# Autodesk Inventor assembly: EngranajesPegados
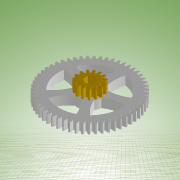
[picture p0: Inventor's stored thumbnail of the model, 180x180]
Saved by Autodesk Inventor 2022 (Build 260153000, 153)
## iProperties
Created: 2022-03-08
Part Number: EngranajesPegados
Document SubType Name: Assembly
Designer: Marco
Author: Marco
## Documents named in this file (3)
- C:\Users\steff\Desktop\9noSemestre\Diseño\MiniProyecto\Archivos STL\EngranajesPegados.iam
- C:\Users\steff\Desktop\9noSemestre\Diseño\MiniProyecto\Engranaje1.ipt
- C:\Users\steff\Desktop\9noSemestre\Diseño\MiniProyecto\Piñon1.ipt
## Components (2 placed, 2 different names)
1. Engranaje1:1 — Coincidencia:1, Coincidencia:2, Coincidencia:3
2. Piñon1:1 — Coincidencia:1, Coincidencia:2, Coincidencia:3
## Relationships (3: Mate 3)
- Coincidencia:1 [Mate]: Engranaje1:1 ↔ Piñon1:1
- Coincidencia:2 [Mate]: Engranaje1:1 ↔ Piñon1:1
- Coincidencia:3 [Mate]: Engranaje1:1 ↔ Piñon1:1
